# Autodesk Inventor assembly: robot
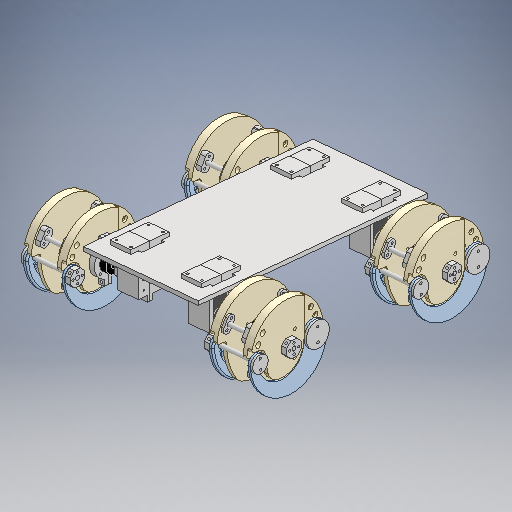
[picture p0: Inventor's stored thumbnail of the model, 512x512]
Saved by Autodesk Inventor 2025.1 (Build 291241000, 241)
## iProperties
Created: 2025-03-25
Part Number: robot
Document SubType Name: Assembly
Designer: 8roke
Author: 8roke
## Documents named in this file (4)
- C:\Users\8roke\OneDrive\문서\Inventor\WheelLegHybridRobot\robot\v1.0\robot.iam
- C:\Users\8roke\OneDrive\문서\Inventor\WheelLegHybridRobot\body\v1.0\body.ipt
- C:\Users\8roke\OneDrive\문서\Inventor\WheelLegHybridRobot\wheel\v3.2\wheel.iam
- C:\Users\8roke\OneDrive\문서\Inventor\WheelLegHybridRobot\wheel\v3.2\wheel_MIR.iam
## Components (5 placed, 3 different names)
1. body:1 — 메이트:1, 메이트:2, 메이트:3, 메이트:4, 메이트:5, 메이트:6, 메이트:7, 메이트:8, 메이트:9, 메이트:10, 메이트:11, 메이트:12, 플러쉬:1, 플러쉬:2, 플러쉬:3, 메이트:13
2. wheel:1 [sub-assembly] — 메이트:1, 메이트:2, 메이트:3
3. wheel:2 [sub-assembly] — 메이트:4, 메이트:5, 메이트:6
4. wheel_MIR:1 [sub-assembly] — 메이트:7, 메이트:8, 메이트:9
5. wheel_MIR:2 [sub-assembly] — 메이트:10, 메이트:11, 메이트:12
## Relationships (16: Mate 13, Flush 3)
- 메이트:1 [Mate]: body:1 ↔ wheel:1
- 메이트:2 [Mate]: body:1 ↔ wheel:1
- 메이트:3 [Mate]: body:1 ↔ wheel:1
- 메이트:4 [Mate]: body:1 ↔ wheel:2
- 메이트:5 [Mate]: body:1 ↔ wheel:2
- 메이트:6 [Mate]: body:1 ↔ wheel:2
- 메이트:7 [Mate]: body:1 ↔ wheel_MIR:1
- 메이트:8 [Mate]: body:1 ↔ wheel_MIR:1
- 메이트:9 [Mate]: body:1 ↔ wheel_MIR:1
- 메이트:10 [Mate]: body:1 ↔ wheel_MIR:2
- 메이트:11 [Mate]: body:1 ↔ wheel_MIR:2
- 메이트:12 [Mate]: body:1 ↔ wheel_MIR:2
- 플러쉬:1 [Flush]: body:1
- 플러쉬:2 [Flush]: body:1
- 플러쉬:3 [Flush]: body:1
- 메이트:13 [Mate]: body:1
